# Autodesk Inventor assembly: Assembly1
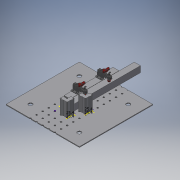
[picture p0: Inventor's stored thumbnail of the model, 180x180]
Saved by Autodesk Inventor 2018 (Build 220112000, 112)
## iProperties
Created: 2018-12-05
Part Number: Assembly1
Document SubType Name: Assembly
Designer: gbgic
Author: gbgic
## Documents named in this file (7)
- C:\Users\s-4009421\Downloads\Drill Jig Assembly v1.iam
- C:\Users\s-4009421\Downloads\Drill Jig Base.ipt
- C:\Users\Gabriel\Documents\GitHub\2019CAD\Tube Beam.ipt
- C:\Users\s-4009421\Downloads\AIS2018\AIS2018\305-U.iam
- C:\Users\s-4009421\Downloads\Jig2.1_1x1_Bolt_Pattern_PIN.ipt
- C:\Users\s-4009421\Downloads\1x1 Beam Test.ipt
- C:\Users\s-4009421\Downloads\Zero Twosday.ipt
## Components (8 placed, 6 different names)
1. Drill Jig Base:1 — Mate:1, Mate:2, Mate:3, Mate:7, Mate:8, Mate:9, Mate:10, Mate:11, Mate:12
2. Tube Beam:1 — Mate:1, Mate:2, Mate:3, Angle:1, Mate:4, Mate:5, Mate:6
3. 305-U:1 [sub-assembly] — Angle:1, Mate:4, Mate:13
4. 305-U:2 [sub-assembly] — Mate:5, Mate:6, Mate:14
5. Jig2.1_1x1_Bolt_Pattern_PIN:1 — Mate:7, Mate:8
6. Jig2.1_1x1_Bolt_Pattern_PIN:2 — Mate:9, Mate:10
7. 1x1 Beam Test:1
8. Zero Twosday:1 — Mate:11, Mate:12, Mate:13, Mate:14
## Relationships (15: Mate 14, Angle 1)
- Mate:1: Drill Jig Base:1 ↔ Tube Beam:1
- Mate:2: Drill Jig Base:1 ↔ Tube Beam:1
- Mate:3: Drill Jig Base:1 ↔ Tube Beam:1
- Angle:1 (0 deg): Tube Beam:1 ↔ 305-U:1
- Mate:4: Tube Beam:1 ↔ 305-U:1
- Mate:5: Tube Beam:1 ↔ 305-U:2
- Mate:6: Tube Beam:1 ↔ 305-U:2
- Mate:7: Drill Jig Base:1 ↔ Jig2.1_1x1_Bolt_Pattern_PIN:1
- Mate:8: Drill Jig Base:1 ↔ Jig2.1_1x1_Bolt_Pattern_PIN:1
- Mate:9: Drill Jig Base:1 ↔ Jig2.1_1x1_Bolt_Pattern_PIN:2
- Mate:10: Drill Jig Base:1 ↔ Jig2.1_1x1_Bolt_Pattern_PIN:2
- Mate:11: Drill Jig Base:1 ↔ Zero Twosday:1
- Mate:12: Drill Jig Base:1 ↔ Zero Twosday:1
- Mate:13: 305-U:1 ↔ Zero Twosday:1
- Mate:14: 305-U:2 ↔ Zero Twosday:1
